# Autodesk Inventor assembly: shooter-v1-roller
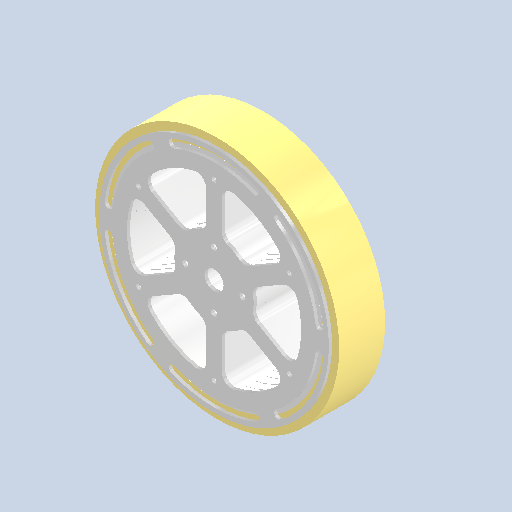
[picture p0: Inventor's stored thumbnail of the model, 512x512]
Saved by Autodesk Inventor 2025.1 (Build 291241000, 241)
## iProperties
Created: 2024-10-12
Part Number: shooter-v1-roller
Document SubType Name: Assembly
Designer: haruy
Author: haruy
## Documents named in this file (5)
- C:\Users\haruy\Documents\ロボコン\NHK2025\cad\nagahisa\shooter\shooter-v1-roller.iam
- C:\Users\haruy\Documents\ロボコン\NHK2025\cad\nagahisa\shooter\TH22_3DP_roller_fixer_sn.ipt
- C:\Users\haruy\Documents\ロボコン\NHK2025\cad\nagahisa\shooter\TH22_AlBoard_roller_sn.ipt
- C:\Users\haruy\Documents\ロボコン\NHK2025\cad\nagahisa\shooter\TH22_POM_roller_sn.ipt
- C:\Users\haruy\Documents\ロボコン\NHK2025\cad\nagahisa\shooter\TH22_Urethane_roller_sn.ipt
## Components (9 placed, 4 different names)
1. TH22_3DP_roller_fixer_sn:1 — 挿入:3
2. TH22_AlBoard_roller_sn:1 — 挿入:2, 挿入:3
3. TH22_POM_roller_sn:1 — 挿入:1, 挿入:2, 挿入:4
4. TH22_Urethane_roller_sn:1 — 挿入:1
5. TH22_POM_roller_sn:2 — 挿入:4, 挿入:5
6. TH22_POM_roller_sn:3 — 挿入:5, 挿入:6
7. TH22_POM_roller_sn:4 — 挿入:6, 挿入:7
8. TH22_POM_roller_sn:5 — 挿入:7, 挿入:8
9. TH22_AlBoard_roller_sn:2 — 挿入:8
## Relationships (8: Insert 8)
- 挿入:1 [Insert]: TH22_POM_roller_sn:1 ↔ TH22_Urethane_roller_sn:1
- 挿入:2 [Insert]: TH22_AlBoard_roller_sn:1 ↔ TH22_POM_roller_sn:1
- 挿入:3 [Insert]: TH22_3DP_roller_fixer_sn:1 ↔ TH22_AlBoard_roller_sn:1
- 挿入:4 [Insert]: TH22_POM_roller_sn:1 ↔ TH22_POM_roller_sn:2
- 挿入:5 [Insert]: TH22_POM_roller_sn:2 ↔ TH22_POM_roller_sn:3
- 挿入:6 [Insert]: TH22_POM_roller_sn:3 ↔ TH22_POM_roller_sn:4
- 挿入:7 [Insert]: TH22_POM_roller_sn:4 ↔ TH22_POM_roller_sn:5
- 挿入:8 [Insert]: TH22_POM_roller_sn:5 ↔ TH22_AlBoard_roller_sn:2
